# Autodesk Inventor assembly: アーム先端ツイン1
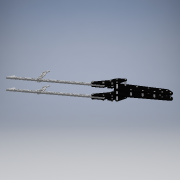
[picture p0: Inventor's stored thumbnail of the model, 180x180]
Saved by Autodesk Inventor 2020 (Build 240168000, 168)
## iProperties
Created: 2018-11-26
Part Number: アーム先端ツイン1
Material: 一般
Document SubType Name: Assembly
Designer: 雪村
Mass: 198.453 g
Surface Area: 903.926 cm^2
Volume: 99.4928 cm^3
Density: 1.99464 g/cm^3
Author: 雪村
## Documents named in this file (18)
- C:\Users\white\Documents\SRDC\SRDC\Inventor_2017\2018年機体\2020年4年機体\アーム先端ツイン1.iam
- C:\Users\white\Documents\SRDC\SRDC\Inventor_2017\2018年機体\パーツ\スペーサーm3,16.ipt
- C:\Users\white\Documents\SRDC\SRDC\Inventor_2017\2018年機体\パーツ\スペーサーm3,4.ipt
- C:\Users\white\Documents\SRDC\SRDC\Inventor_2017\2018年機体\パーツ\ネジ鍋m3,18.ipt
- C:\Users\white\Documents\SRDC\SRDC\Inventor_2017\2018年機体\パーツ\ナイロンナットm3.ipt
- C:\Users\white\Documents\SRDC\SRDC\Inventor_2017\2018年機体\パーツ\ネジ鍋m3,08.ipt
- C:\Users\white\Documents\SRDC\SRDC\Inventor_2017\2018年機体\パーツ\スペーサーm3,18.ipt
- C:\Users\white\Documents\SRDC\SRDC\Inventor_2017\2018年機体\2020年4年機体\アーム抑えツイン1.ipt
- C:\Users\white\Documents\SRDC\SRDC\Inventor_2017\2018年機体\パーツ\オイレスフランジ付き06080312.ipt
- C:\Users\white\Documents\SRDC\SRDC\Inventor_2017\2018年機体\パーツ\スペーサーm3,7.ipt
- C:\Users\white\Documents\SRDC\SRDC\Inventor_2017\2018年機体\パーツ\ネジ鍋m3,30.ipt
- C:\Users\white\Documents\SRDC\SRDC\Inventor_2017\2018年機体\2020年4年機体\アーム先端第1関節2.1.ipt
- C:\Users\white\Documents\SRDC\SRDC\Inventor_2017\2018年機体\2020年4年機体\アーム先端第1関節2.1_MIR.ipt
- C:\Users\white\Documents\SRDC\SRDC\Inventor_2017\2018年機体\2020年4年機体\アーム先端1.ipt
- C:\Users\white\Documents\SRDC\SRDC\Inventor_2017\2018年機体\2020年4年機体\アーム先端返し1.ipt
- C:\Users\white\Documents\SRDC\SRDC\Inventor_2017\2018年機体\2020年4年機体\アーム先端返し抑え1.ipt
- C:\Users\white\Documents\SRDC\SRDC\Inventor_2017\2018年機体\2020年4年機体\アーム先端ポリカパーツ1.ipt
- C:\Users\white\Documents\SRDC\SRDC\Inventor_2017\2018年機体\2020年4年機体\アーム先端ポリカパーツ1_MIR.ipt
## Components (78 placed, 17 different names)
1. アーム先端第1関節2.1:1 — 挿入:37, 挿入:38, 挿入:39, 挿入:43, 挿入:44, 挿入:46, 挿入:47, 挿入:48, 挿入:49, 挿入:50, 挿入:51, 挿入:184, 挿入:185, 挿入:186, 挿入:187, 挿入:208
2. アーム先端1:2 — 挿入:131, メイト:3, 挿入:132, メイト:4, 挿入:204, 正接:2
3. スペーサーm3,16:1 — 挿入:208
4. スペーサーm3,16:2 — 挿入:48
5. スペーサーm3,4:1 — 挿入:126
6. スペーサーm3,4:2 — 挿入:125
7. ネジ鍋m3,18:1 — 挿入:136
8. ネジ鍋m3,18:2 — 挿入:133
9. ネジ鍋m3,18:3 — 挿入:135
10. ネジ鍋m3,18:4 — 挿入:134
11. ナイロンナットm3:1 — 挿入:127
12. ナイロンナットm3:2 — 挿入:130, メイト:3
13. ナイロンナットm3:3 — 挿入:128
14. ナイロンナットm3:4 — 挿入:129
15. スペーサーm3,16:3 — 挿入:184
16. スペーサーm3,16:5
17. スペーサーm3,16:6
18. スペーサーm3,16:7
19. スペーサーm3,16:8
20. スペーサーm3,16:9 — 挿入:47
21. スペーサーm3,16:10
22. ネジ鍋m3,08:1
23. ネジ鍋m3,08:2
24. ネジ鍋m3,08:3
25. ネジ鍋m3,08:6 — 挿入:38
26. ネジ鍋m3,08:8
27. ネジ鍋m3,08:9
28. ネジ鍋m3,08:10
29. ネジ鍋m3,08:12 — 挿入:37
30. ネジ鍋m3,08:14 — 挿入:39
31. ネジ鍋m3,08:17 — 挿入:43
32. ネジ鍋m3,08:19 — 挿入:44
33. ネジ鍋m3,08:21 — 挿入:46
34. スペーサーm3,18:1 — 挿入:51
35. スペーサーm3,18:2 — 挿入:209
36. スペーサーm3,18:3 — 挿入:50, 挿入:75
37. スペーサーm3,18:4 — 挿入:49, 挿入:73, 挿入:76
38. スペーサーm3,18:5 — 挿入:78
39. スペーサーm3,18:6 — 挿入:74, 挿入:77
40. アーム抑えツイン1:1 — 挿入:75, 挿入:76, 挿入:194, 挿入:195, 挿入:196
41. アーム抑えツイン1:2 — 挿入:77, 挿入:78, 挿入:191, 挿入:192, 挿入:193, 挿入:209
42. アーム先端1:1 — 挿入:154, 挿入:155, 挿入:156, 挿入:205, 正接:1
43. スペーサーm3,4:3 — 挿入:158, 挿入:163
44. オイレスフランジ付き06080312:1 — 挿入:73, 挿入:138
45. オイレスフランジ付き06080312:2 — 挿入:168
46. オイレスフランジ付き06080312:3 — 挿入:74, 挿入:169
47. オイレスフランジ付き06080312:4 — 挿入:137
48. ネジ鍋m3,18:5 — 挿入:162
49. ネジ鍋m3,18:6 — 挿入:159
50. ネジ鍋m3,18:7 — 挿入:160
51. ネジ鍋m3,18:8 — 挿入:161
52. ナイロンナットm3:5 — 挿入:164
53. ナイロンナットm3:6 — 挿入:167
54. ナイロンナットm3:7 — 挿入:165
55. ナイロンナットm3:8 — 挿入:166
56. アーム先端ポリカパーツ1:1 — 挿入:125, 挿入:126, 挿入:127, 挿入:128, 挿入:129, 挿入:130, 挿入:131, 挿入:138
57. アーム先端ポリカパーツ1:2 — 挿入:154, 挿入:155, 挿入:158, 挿入:159, 挿入:160, 挿入:161, 挿入:162, 挿入:168
58. アーム先端ポリカパーツ1_MIR:1 — 挿入:156, 挿入:163, 挿入:164, 挿入:165, 挿入:166, 挿入:167, 挿入:169
59. アーム先端ポリカパーツ1_MIR:2 — 挿入:132, メイト:4, 挿入:133, 挿入:134, 挿入:135, 挿入:136, 挿入:137
60. アーム先端第1関節2.1_MIR:1
61. ネジ鍋m3,08:22 — 挿入:187
62. ネジ鍋m3,08:23
63. ネジ鍋m3,08:24 — 挿入:186
64. ネジ鍋m3,08:25
65. ネジ鍋m3,08:26
66. ネジ鍋m3,08:27 — 挿入:185
67. ネジ鍋m3,30:1 — 挿入:193
68. ネジ鍋m3,30:2 — 挿入:191
69. ネジ鍋m3,30:3 — 挿入:192
70. ネジ鍋m3,30:4 — 挿入:194
71. ネジ鍋m3,30:5 — 挿入:195
72. ネジ鍋m3,30:6 — 挿入:196
73. アーム先端返し1:1 — 挿入:202, メイト:6, 挿入:204
74. アーム先端返し1:2 — 挿入:200, メイト:7, 挿入:205
75. アーム先端返し抑え1:1 — 挿入:199, メイト:7
76. アーム先端返し抑え1:2 — 挿入:201, メイト:6
77. スペーサーm3,7:1 — 挿入:199, 挿入:200, 正接:1
78. スペーサーm3,7:2 — 挿入:201, 挿入:202, 正接:2
## Relationships (84: Insert 78, Mate 4, Tangent 2)
- 挿入:37 [Insert]: アーム先端第1関節2.1:1 ↔ ネジ鍋m3,08:12
- 挿入:38 [Insert]: アーム先端第1関節2.1:1 ↔ ネジ鍋m3,08:6
- 挿入:39 [Insert]: アーム先端第1関節2.1:1 ↔ ネジ鍋m3,08:14
- 挿入:43 [Insert]: アーム先端第1関節2.1:1 ↔ ネジ鍋m3,08:17
- 挿入:44 [Insert]: アーム先端第1関節2.1:1 ↔ ネジ鍋m3,08:19
- 挿入:46 [Insert]: アーム先端第1関節2.1:1 ↔ ネジ鍋m3,08:21
- 挿入:47 [Insert]: アーム先端第1関節2.1:1 ↔ スペーサーm3,16:9
- 挿入:48 [Insert]: アーム先端第1関節2.1:1 ↔ スペーサーm3,16:2
- 挿入:49 [Insert]: アーム先端第1関節2.1:1 ↔ スペーサーm3,18:4
- 挿入:50 [Insert]: アーム先端第1関節2.1:1 ↔ スペーサーm3,18:3
- 挿入:51 [Insert]: アーム先端第1関節2.1:1 ↔ スペーサーm3,18:1
- 挿入:73 [Insert]: スペーサーm3,18:4 ↔ オイレスフランジ付き06080312:1
- 挿入:74 [Insert]: スペーサーm3,18:6 ↔ オイレスフランジ付き06080312:3
- 挿入:75 [Insert]: スペーサーm3,18:3 ↔ アーム抑えツイン1:1
- 挿入:76 [Insert]: スペーサーm3,18:4 ↔ アーム抑えツイン1:1
- 挿入:77 [Insert]: スペーサーm3,18:6 ↔ アーム抑えツイン1:2
- 挿入:78 [Insert]: スペーサーm3,18:5 ↔ アーム抑えツイン1:2
- 挿入:125 [Insert]: スペーサーm3,4:2 ↔ アーム先端ポリカパーツ1:1
- 挿入:126 [Insert]: スペーサーm3,4:1 ↔ アーム先端ポリカパーツ1:1
- 挿入:127 [Insert]: ナイロンナットm3:1 ↔ アーム先端ポリカパーツ1:1
- 挿入:128 [Insert]: ナイロンナットm3:3 ↔ アーム先端ポリカパーツ1:1
- 挿入:129 [Insert]: ナイロンナットm3:4 ↔ アーム先端ポリカパーツ1:1
- 挿入:130 [Insert]: ナイロンナットm3:2 ↔ アーム先端ポリカパーツ1:1
- 挿入:131 [Insert]: アーム先端1:2 ↔ アーム先端ポリカパーツ1:1
- メイト:3 [Mate]: アーム先端1:2 ↔ ナイロンナットm3:2
- 挿入:132 [Insert]: アーム先端1:2 ↔ アーム先端ポリカパーツ1_MIR:2
- メイト:4 [Mate]: アーム先端1:2 ↔ アーム先端ポリカパーツ1_MIR:2
- 挿入:133 [Insert]: ネジ鍋m3,18:2 ↔ アーム先端ポリカパーツ1_MIR:2
- 挿入:134 [Insert]: ネジ鍋m3,18:4 ↔ アーム先端ポリカパーツ1_MIR:2
- 挿入:135 [Insert]: ネジ鍋m3,18:3 ↔ アーム先端ポリカパーツ1_MIR:2
- 挿入:136 [Insert]: ネジ鍋m3,18:1 ↔ アーム先端ポリカパーツ1_MIR:2
- 挿入:137 [Insert]: オイレスフランジ付き06080312:4 ↔ アーム先端ポリカパーツ1_MIR:2
- 挿入:138 [Insert]: オイレスフランジ付き06080312:1 ↔ アーム先端ポリカパーツ1:1
- 挿入:154 [Insert]: アーム先端1:1 ↔ アーム先端ポリカパーツ1:2
- 挿入:155 [Insert]: アーム先端1:1 ↔ アーム先端ポリカパーツ1:2
- 挿入:156 [Insert]: アーム先端1:1 ↔ アーム先端ポリカパーツ1_MIR:1
- 挿入:158 [Insert]: スペーサーm3,4:3 ↔ アーム先端ポリカパーツ1:2
- 挿入:159 [Insert]: ネジ鍋m3,18:6 ↔ アーム先端ポリカパーツ1:2
- 挿入:160 [Insert]: ネジ鍋m3,18:7 ↔ アーム先端ポリカパーツ1:2
- 挿入:161 [Insert]: ネジ鍋m3,18:8 ↔ アーム先端ポリカパーツ1:2
- 挿入:162 [Insert]: ネジ鍋m3,18:5 ↔ アーム先端ポリカパーツ1:2
- 挿入:163 [Insert]: スペーサーm3,4:3 ↔ アーム先端ポリカパーツ1_MIR:1
- 挿入:164 [Insert]: ナイロンナットm3:5 ↔ アーム先端ポリカパーツ1_MIR:1
- 挿入:165 [Insert]: ナイロンナットm3:7 ↔ アーム先端ポリカパーツ1_MIR:1
- 挿入:166 [Insert]: ナイロンナットm3:8 ↔ アーム先端ポリカパーツ1_MIR:1
- 挿入:167 [Insert]: ナイロンナットm3:6 ↔ アーム先端ポリカパーツ1_MIR:1
- 挿入:168 [Insert]: オイレスフランジ付き06080312:2 ↔ アーム先端ポリカパーツ1:2
- 挿入:169 [Insert]: オイレスフランジ付き06080312:3 ↔ アーム先端ポリカパーツ1_MIR:1
- [Insert]: スペーサーm3,16:3 ↔ アーム先端第1関節2.1_MIR:1
- [Insert]: スペーサーm3,16:8 ↔ アーム先端第1関節2.1_MIR:1
- [Insert]: ネジ鍋m3,08:10 ↔ アーム先端第1関節2.1_MIR:1
- [Insert]: ネジ鍋m3,08:9 ↔ アーム先端第1関節2.1_MIR:1
- [Insert]: ネジ鍋m3,08:3 ↔ アーム先端第1関節2.1_MIR:1
- [Insert]: ネジ鍋m3,08:2 ↔ アーム先端第1関節2.1_MIR:1
- [Insert]: ネジ鍋m3,08:8 ↔ アーム先端第1関節2.1_MIR:1
- [Insert]: ネジ鍋m3,08:1 ↔ アーム先端第1関節2.1_MIR:1
- [Insert]: スペーサーm3,18:6 ↔ アーム先端第1関節2.1_MIR:1
- [Insert]: スペーサーm3,18:5 ↔ アーム先端第1関節2.1_MIR:1
- [Insert]: スペーサーm3,16:2 ↔ アーム先端第1関節2.1_MIR:1
- 挿入:184 [Insert]: アーム先端第1関節2.1:1 ↔ スペーサーm3,16:3
- 挿入:185 [Insert]: アーム先端第1関節2.1:1 ↔ ネジ鍋m3,08:27
- 挿入:186 [Insert]: アーム先端第1関節2.1:1 ↔ ネジ鍋m3,08:24
- 挿入:187 [Insert]: アーム先端第1関節2.1:1 ↔ ネジ鍋m3,08:22
- [Insert]: アーム先端第1関節2.1_MIR:1 ↔ ネジ鍋m3,08:25
- [Insert]: アーム先端第1関節2.1_MIR:1 ↔ ネジ鍋m3,08:23
- [Insert]: アーム先端第1関節2.1_MIR:1 ↔ ネジ鍋m3,08:26
- 挿入:191 [Insert]: アーム抑えツイン1:2 ↔ ネジ鍋m3,30:2
- 挿入:192 [Insert]: アーム抑えツイン1:2 ↔ ネジ鍋m3,30:3
- 挿入:193 [Insert]: アーム抑えツイン1:2 ↔ ネジ鍋m3,30:1
- 挿入:194 [Insert]: アーム抑えツイン1:1 ↔ ネジ鍋m3,30:4
- 挿入:195 [Insert]: アーム抑えツイン1:1 ↔ ネジ鍋m3,30:5
- 挿入:196 [Insert]: アーム抑えツイン1:1 ↔ ネジ鍋m3,30:6
- 挿入:199 [Insert]: アーム先端返し抑え1:1 ↔ スペーサーm3,7:1
- 挿入:200 [Insert]: アーム先端返し1:2 ↔ スペーサーm3,7:1
- 挿入:201 [Insert]: アーム先端返し抑え1:2 ↔ スペーサーm3,7:2
- 挿入:202 [Insert]: アーム先端返し1:1 ↔ スペーサーm3,7:2
- メイト:6 [Mate]: アーム先端返し1:1 ↔ アーム先端返し抑え1:2
- メイト:7 [Mate]: アーム先端返し1:2 ↔ アーム先端返し抑え1:1
- 挿入:204 [Insert]: アーム先端1:2 ↔ アーム先端返し1:1
- 挿入:205 [Insert]: アーム先端1:1 ↔ アーム先端返し1:2
- 正接:1 [Tangent]: アーム先端1:1 ↔ スペーサーm3,7:1
- 正接:2 [Tangent]: アーム先端1:2 ↔ スペーサーm3,7:2
- 挿入:208 [Insert]: アーム先端第1関節2.1:1 ↔ スペーサーm3,16:1
- 挿入:209 [Insert]: スペーサーm3,18:2 ↔ アーム抑えツイン1:2
